# Autodesk Inventor assembly: Left side arm
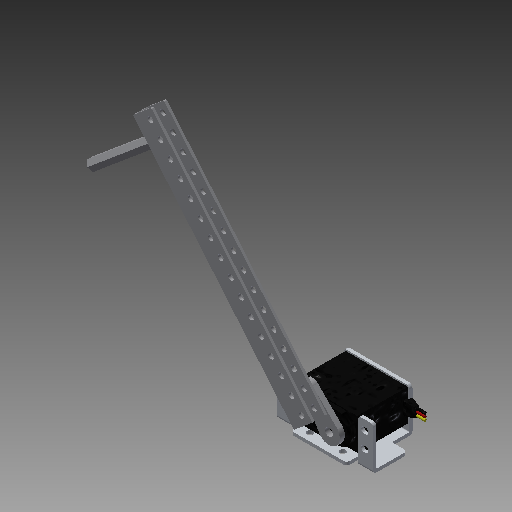
[picture p0: Inventor's stored thumbnail of the model, 512x512]
Saved by Autodesk Inventor 2019 (Build 230136000, 136)
## iProperties
Created: 2020-02-15
Part Number: Left side arm
Document SubType Name: Assembly
Designer: Delta
Author: Delta
## Documents named in this file (6)
- C:\Robotics\2019-20_CAD\offseason\Left side arm.iam
- C:\Robotics\COTSParts\Tetrix\39060_txm-standard servo bracket.ipt
- C:\Robotics\COTSParts\Tetrix\Tetrix 180 Servo.ipt
- C:\Robotics\2019-20_CAD\Collection\Servo horn.ipt
- C:\Robotics\2019-20_CAD\Drive Train\585392MiniChannel6.31in.ipt
- C:\Robotics\COTSParts\Tetrix\Hex standoff 2in.ipt
## Components (5 placed, 5 different names)
1. 39060_txm-standard servo bracket:1 — Mate:1, Mate:2, Angle:1
2. Tetrix 180 Servo:1 — Mate:1, Mate:2, Angle:1, Mate:3, Mate:4
3. Servo horn:1 — Mate:3, Mate:4, Mate:5, Mate:6, Angle:2
4. 585392MiniChannel6.31in:1 — Mate:5, Mate:6, Angle:2, Mate:7, Mate:8
5. Hex standoff 2in:1 — Mate:7, Mate:8
## Relationships (10: Mate 8, Angle 2)
- Mate:1: 39060_txm-standard servo bracket:1 ↔ Tetrix 180 Servo:1
- Mate:2: 39060_txm-standard servo bracket:1 ↔ Tetrix 180 Servo:1
- Angle:1 (0 deg): 39060_txm-standard servo bracket:1 ↔ Tetrix 180 Servo:1
- Mate:3: Tetrix 180 Servo:1 ↔ Servo horn:1
- Mate:4: Tetrix 180 Servo:1 ↔ Servo horn:1
- Mate:5: Servo horn:1 ↔ 585392MiniChannel6.31in:1
- Mate:6: Servo horn:1 ↔ 585392MiniChannel6.31in:1
- Angle:2 (185 deg): Servo horn:1 ↔ 585392MiniChannel6.31in:1
- Mate:7: 585392MiniChannel6.31in:1 ↔ Hex standoff 2in:1
- Mate:8: 585392MiniChannel6.31in:1 ↔ Hex standoff 2in:1
